# Autodesk Inventor assembly: 276-2174
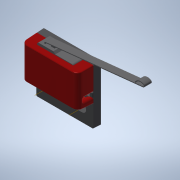
[picture p0: Inventor's stored thumbnail of the model, 180x180]
Saved by Autodesk Inventor 2020 (Build 240168000, 168)
## iProperties
Created: 2012-04-10
Part Number: 276-2174
Document SubType Name: Assembly
Catalog Web Link: http://www.vexrobotics.com/products/accessories/sensors/276-2174.html
Vendor: VEX
Designer: Autodesk Inc.
Category: Sensors
Company: Autodesk Inc.
Author: Autodesk Inc.
## Documents named in this file (4)
- D:\Valut\ncrCadLib\传感器\Limit Switch.iam
- D:\Valut\ncrCadLib\传感器\Reference Parts\LIMIT-SWITCH-MICROSWITCH.ipt
- D:\Valut\ncrCadLib\传感器\Reference Parts\LIMIT-SWITCH-BOTTOM.ipt
- D:\Valut\ncrCadLib\传感器\Reference Parts\LIMIT-SWITCH-TOP.ipt
## Components (3 placed, 3 different names)
1. LIMIT-SWITCH-MICROSWITCH:1 — Mate:5, Mate:6, Mate:7
2. LIMIT-SWITCH-BOTTOM:1 — Mate:1, Mate:2, Insert:1, Insert:2, Mate:5, Mate:6, Mate:7
3. LIMIT-SWITCH-TOP:1 — Insert:1, Insert:2
## Relationships (9: Mate 7, Insert 2)
- Mate:1: LIMIT-SWITCH-BOTTOM:1
- Mate:2: LIMIT-SWITCH-BOTTOM:1
- Mate:3
- Mate:4
- Insert:1: LIMIT-SWITCH-BOTTOM:1 ↔ LIMIT-SWITCH-TOP:1
- Insert:2: LIMIT-SWITCH-BOTTOM:1 ↔ LIMIT-SWITCH-TOP:1
- Mate:5: LIMIT-SWITCH-MICROSWITCH:1 ↔ LIMIT-SWITCH-BOTTOM:1
- Mate:6: LIMIT-SWITCH-MICROSWITCH:1 ↔ LIMIT-SWITCH-BOTTOM:1
- Mate:7: LIMIT-SWITCH-MICROSWITCH:1 ↔ LIMIT-SWITCH-BOTTOM:1
